# Autodesk Inventor assembly: Bearing
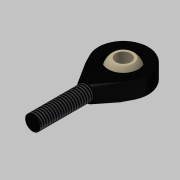
[picture p0: Inventor's stored thumbnail of the model, 180x180]
Saved by Autodesk Inventor 2015 SP1 (Build 190203100, 203)
## iProperties
Created: 2014-07-13
Part Number: Bearing
Document SubType Name: Assembly
Designer: User
Author: User
## Documents named in this file (3)
- C:\Users\Val\Desktop\ExoGit\elysium-max-exoskeleton\src\External\Bearing.iam
- C:\Users\Val\Desktop\ExoGit\elysium-max-exoskeleton\src\External\BearingBall.ipt
- C:\Users\Val\Desktop\ExoGit\elysium-max-exoskeleton\src\External\BearingBody.ipt
## Components (2 placed, 2 different names)
1. Ball — Mate:1, Angle:1
2. Body — Mate:1, Angle:1
## Relationships (2: Mate 1, Angle 1)
- Mate:1: Ball ↔ Body
- Angle:1 (0 deg): Ball ↔ Body
